# Autodesk Inventor assembly: AngleJoint
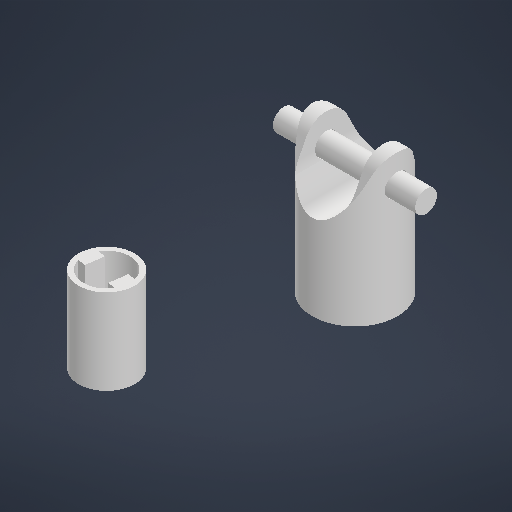
[picture p0: Inventor's stored thumbnail of the model, 512x512]
Saved by Autodesk Inventor 2026.2 (Build 302298010, 298A)
## iProperties
Created: 2026-06-25
Part Number: AngleJoint
Document SubType Name: Assembly
Designer: frede
Author: frede
## Documents named in this file (4)
- C:\Git\AppliedAutomationProject\CAD\feeder\AngleJoint\AngleJoint.iam
- C:\Git\AppliedAutomationProject\CAD\feeder\AngleJoint\Base_joint.ipt
- C:\Git\AppliedAutomationProject\CAD\feeder\Axel_connector.ipt
- C:\Git\AppliedAutomationProject\CAD\feeder\AngleJoint\MiddleJoint.ipt
## Components (3 placed, 3 different names)
1. Base_joint:1 — Mate:1
2. Axel_connector:1
3. MiddleJoint:1 — Mate:1
## Relationships (1: Mate 1)
- Mate:1: Base_joint:1 ↔ MiddleJoint:1
